# Autodesk Inventor assembly: BoschCollector
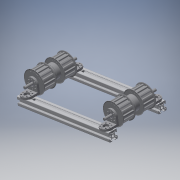
[picture p0: Inventor's stored thumbnail of the model, 180x180]
Saved by Autodesk Inventor 2016 (Build 200138000, 138)
## iProperties
Created: 2016-10-28
Part Number: BoschCollector
Document SubType Name: Assembly
Designer: Delta
Author: Delta
## Documents named in this file (12)
- C:\Robotics\CAD\2016-17_CAD\BoschCollector.iam
- C:\Robotics\CAD\COTSParts\Brecoflex\ls40t10_15-2_hub-32x10_d-8h7.ipt
- C:\Robotics\CAD\COTSParts\Actobotics\545 parts\545400.ipt
- C:\Robotics\CAD\COTSParts\Bearings - AndyMark\Bearing 250 ID 500 OD flanged.ipt
- C:\Robotics\CAD\COTSParts\Bosch Extrusion\Bosch 20x20 9 in actual.ipt
- C:\Robotics\CAD\COTSParts\Bosch Extrusion\6mm block nut M4.ipt
- C:\Robotics\CAD\COTSParts\Brecoflex\ls40t10_15-2_hub-32x10_d-8h7_MIR.ipt
- C:\Robotics\CAD\COTSParts\Actobotics\545 parts\545400_MIR.ipt
- C:\Robotics\CAD\COTSParts\Bearings - AndyMark\Bearing 250 ID 500 OD flanged_MIR.ipt
- C:\Robotics\CAD\COTSParts\Bosch Extrusion\Bosch 20x20 9 in actual_MIR.ipt
- C:\Robotics\CAD\COTSParts\Bosch Extrusion\6mm block nut M4_MIR.ipt
- C:\Robotics\CAD\COTSParts\Actobotics\634 parts\634082.ipt
## Components (24 placed, 11 different names)
1. ls40t10_15-2_hub-32x10_d-8h7:2 — Insert:5
2. 545400:1 — Insert:4, Insert:8, Insert:9
3. Bearing 250 ID 500 OD flanged:1 — Insert:4, Insert:5
4. Bosch 20x20 9 in actual:1 — Mate:1, Mate:2, Flush:1, Mate:3, Mate:4, Mate:9, Mate:10, Mate:11, Flush:4, Mate:12
5. 6mm block nut M4:1 — Mate:1, Mate:4, Insert:8
6. 6mm block nut M4:2 — Mate:2, Flush:1, Mate:3, Insert:9
7. ls40t10_15-2_hub-32x10_d-8h7_MIR:1 — Insert:10
8. Bearing 250 ID 500 OD flanged_MIR:1 — Insert:10, Insert:11
9. 545400_MIR:1 — Insert:11, Insert:12, Insert:13, Insert:23
10. Bosch 20x20 9 in actual_MIR:1 — Mate:5, Mate:6, Mate:7, Flush:3, Mate:8, Mate:13, Mate:14, Mate:15, Flush:5, Mate:16
11. 6mm block nut M4_MIR:1 — Insert:12, Mate:5, Mate:6
12. 6mm block nut M4_MIR:2 — Insert:13, Mate:7, Flush:3, Mate:8
13. 6mm block nut M4:3 — Mate:9, Mate:10, Insert:15
14. 6mm block nut M4:4 — Mate:11, Flush:4, Mate:12, Insert:14
15. 545400:2 — Insert:14, Insert:15, Insert:16, Insert:22
16. Bearing 250 ID 500 OD flanged:2 — Insert:16, Insert:17
17. ls40t10_15-2_hub-32x10_d-8h7:3 — Insert:17
18. 6mm block nut M4:5 — Mate:13, Mate:14, Insert:19
19. 6mm block nut M4:6 — Mate:15, Flush:5, Mate:16, Insert:18
20. 545400:3 — Insert:18, Insert:19, Insert:20
21. Bearing 250 ID 500 OD flanged_MIR:2 — Insert:20, Insert:21
22. ls40t10_15-2_hub-32x10_d-8h7_MIR:2 — Insert:21
23. 634082:2 — Insert:22
24. 634082:3 — Insert:23
## Relationships (38: Insert 18, Mate 16, Flush 4)
- Insert:4: 545400:1 ↔ Bearing 250 ID 500 OD flanged:1
- Insert:5: ls40t10_15-2_hub-32x10_d-8h7:2 ↔ Bearing 250 ID 500 OD flanged:1
- Mate:1: Bosch 20x20 9 in actual:1 ↔ 6mm block nut M4:1
- Mate:2: Bosch 20x20 9 in actual:1 ↔ 6mm block nut M4:2
- Flush:1: Bosch 20x20 9 in actual:1 ↔ 6mm block nut M4:2
- Mate:3: Bosch 20x20 9 in actual:1 ↔ 6mm block nut M4:2
- Mate:4: Bosch 20x20 9 in actual:1 ↔ 6mm block nut M4:1
- Insert:8: 545400:1 ↔ 6mm block nut M4:1
- Insert:9: 545400:1 ↔ 6mm block nut M4:2
- Insert:10: ls40t10_15-2_hub-32x10_d-8h7_MIR:1 ↔ Bearing 250 ID 500 OD flanged_MIR:1
- Insert:11: Bearing 250 ID 500 OD flanged_MIR:1 ↔ 545400_MIR:1
- Insert:12: 545400_MIR:1 ↔ 6mm block nut M4_MIR:1
- Mate:5: Bosch 20x20 9 in actual_MIR:1 ↔ 6mm block nut M4_MIR:1
- Mate:6: Bosch 20x20 9 in actual_MIR:1 ↔ 6mm block nut M4_MIR:1
- Insert:13: 545400_MIR:1 ↔ 6mm block nut M4_MIR:2
- Mate:7: Bosch 20x20 9 in actual_MIR:1 ↔ 6mm block nut M4_MIR:2
- Flush:3: Bosch 20x20 9 in actual_MIR:1 ↔ 6mm block nut M4_MIR:2
- Mate:8: Bosch 20x20 9 in actual_MIR:1 ↔ 6mm block nut M4_MIR:2
- Mate:9: Bosch 20x20 9 in actual:1 ↔ 6mm block nut M4:3
- Mate:10: Bosch 20x20 9 in actual:1 ↔ 6mm block nut M4:3
- Mate:11: Bosch 20x20 9 in actual:1 ↔ 6mm block nut M4:4
- Flush:4: Bosch 20x20 9 in actual:1 ↔ 6mm block nut M4:4
- Mate:12: Bosch 20x20 9 in actual:1 ↔ 6mm block nut M4:4
- Insert:14: 6mm block nut M4:4 ↔ 545400:2
- Insert:15: 6mm block nut M4:3 ↔ 545400:2
- Insert:16: 545400:2 ↔ Bearing 250 ID 500 OD flanged:2
- Insert:17: Bearing 250 ID 500 OD flanged:2 ↔ ls40t10_15-2_hub-32x10_d-8h7:3
- Mate:13: Bosch 20x20 9 in actual_MIR:1 ↔ 6mm block nut M4:5
- Mate:14: Bosch 20x20 9 in actual_MIR:1 ↔ 6mm block nut M4:5
- Mate:15: Bosch 20x20 9 in actual_MIR:1 ↔ 6mm block nut M4:6
- Flush:5: Bosch 20x20 9 in actual_MIR:1 ↔ 6mm block nut M4:6
- Mate:16: Bosch 20x20 9 in actual_MIR:1 ↔ 6mm block nut M4:6
- Insert:18: 6mm block nut M4:6 ↔ 545400:3
- Insert:19: 6mm block nut M4:5 ↔ 545400:3
- Insert:20: 545400:3 ↔ Bearing 250 ID 500 OD flanged_MIR:2
- Insert:21: Bearing 250 ID 500 OD flanged_MIR:2 ↔ ls40t10_15-2_hub-32x10_d-8h7_MIR:2
- Insert:22 (-18.034 mm): 545400:2 ↔ 634082:2
- Insert:23 (-18.034 mm): 545400_MIR:1 ↔ 634082:3
